# Autodesk Inventor assembly: A2017_T5_02
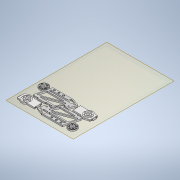
[picture p0: Inventor's stored thumbnail of the model, 180x180]
Saved by Autodesk Inventor 2020 (Build 240168000, 168)
## iProperties
Created: 2021-08-27
Part Number: A2017_T5_02
Document SubType Name: Assembly
Designer: Masato
Author: Masato
## Documents named in this file (5)
- C:\Users\naoki\Documents\Inventor\CitBrains\git_clone\OpenPlatform4_0\コックピット\OpenPlatform_ver3_0\cam\A2017_T5_02.iam
- C:\Users\naoki\Documents\Inventor\CitBrains\git_clone\OpenPlatform4_0\再切削\OpenPlatform_ver3_0\cam\Disposable_Board.ipt
- C:\Users\naoki\Documents\Inventor\CitBrains\git_clone\OpenPlatform4_0\コックピット\OpenPlatform_ver3_0\LowerBody\Leg_joit\Leg_joint_yaw_frame.ipt
- C:\Users\naoki\Documents\Inventor\CitBrains\git_clone\OpenPlatform4_0\コックピット\OpenPlatform_ver3_0\UpperBody\Trunk\Inner_support_stand.ipt
- C:\Users\naoki\Documents\Inventor\CitBrains\git_clone\OpenPlatform4_0\コックピット\OpenPlatform_ver3_0\UpperBody\Trunk\Trunk_lower_flank_frame.ipt
## Components (7 placed, 4 different names)
1. Disposable_Board:1 — メイト:2, メイト:1, フラッシュ:1, フラッシュ:2, 角度:1, フラッシュ:3, 正接:1, フラッシュ:4, 正接:5, 正接:8
2. Leg_joint_yaw_frame:1 — メイト:7, 角度:1, 角度:2, 正接:3, 正接:4
3. Leg_joint_yaw_frame:2 — メイト:10, 角度:2, フラッシュ:3, 正接:1, 正接:2
4. Inner_support_stand:1 — メイト:5, 正接:7, 正接:8
5. Inner_support_stand:2 — メイト:4, 正接:5, 正接:6
6. Trunk_lower_flank_frame:1 — メイト:9, メイト:11, メイト:12, 正接:3, 正接:7
7. Trunk_lower_flank_frame:2 — メイト:8, メイト:11, メイト:12, フラッシュ:4, 正接:2, 正接:4, 正接:6
## Relationships (24: Mate 10, Tangent 8, Flush 4, Angle 2)
- メイト:2 [Mate]: Disposable_Board:1
- メイト:1 [Mate]: Disposable_Board:1
- フラッシュ:1 [Flush]: Disposable_Board:1
- フラッシュ:2 [Flush]: Disposable_Board:1
- メイト:4 [Mate]: Inner_support_stand:2
- メイト:5 [Mate]: Inner_support_stand:1
- メイト:7 [Mate]: Leg_joint_yaw_frame:1
- メイト:8 [Mate]: Trunk_lower_flank_frame:2
- メイト:9 [Mate]: Trunk_lower_flank_frame:1
- メイト:10 [Mate]: Leg_joint_yaw_frame:2
- 角度:1 [Angle] (0 deg): Disposable_Board:1 ↔ Leg_joint_yaw_frame:1
- 角度:2 [Angle] (180 deg): Leg_joint_yaw_frame:1 ↔ Leg_joint_yaw_frame:2
- メイト:11 [Mate] (2.5 mm): Trunk_lower_flank_frame:1 ↔ Trunk_lower_flank_frame:2
- メイト:12 [Mate] (2.5 mm): Trunk_lower_flank_frame:1 ↔ Trunk_lower_flank_frame:2
- フラッシュ:3 [Flush] (2 mm): Disposable_Board:1 ↔ Leg_joint_yaw_frame:2
- 正接:1 [Tangent] (2 mm): Disposable_Board:1 ↔ Leg_joint_yaw_frame:2
- フラッシュ:4 [Flush] (2 mm): Disposable_Board:1 ↔ Trunk_lower_flank_frame:2
- 正接:2 [Tangent] (2.5 mm): Leg_joint_yaw_frame:2 ↔ Trunk_lower_flank_frame:2
- 正接:3 [Tangent] (2.5 mm): Leg_joint_yaw_frame:1 ↔ Trunk_lower_flank_frame:1
- 正接:4 [Tangent] (2.5 mm): Leg_joint_yaw_frame:1 ↔ Trunk_lower_flank_frame:2
- 正接:5 [Tangent] (2 mm): Disposable_Board:1 ↔ Inner_support_stand:2
- 正接:6 [Tangent] (2 mm): Inner_support_stand:2 ↔ Trunk_lower_flank_frame:2
- 正接:7 [Tangent] (2.5 mm): Inner_support_stand:1 ↔ Trunk_lower_flank_frame:1
- 正接:8 [Tangent] (2 mm): Disposable_Board:1 ↔ Inner_support_stand:1
